# Autodesk Inventor assembly: ensamblaje socket
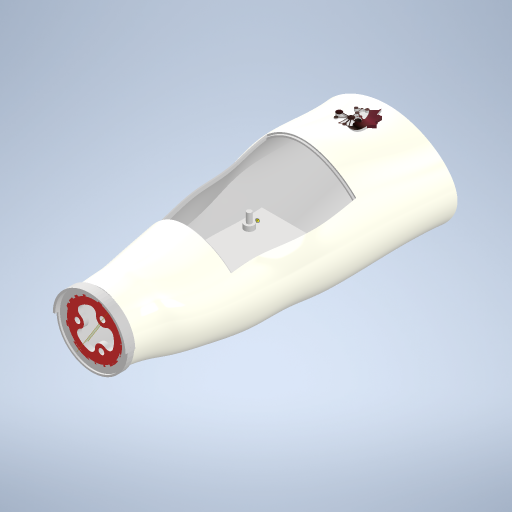
[picture p0: Inventor's stored thumbnail of the model, 512x512]
Saved by Autodesk Inventor 2024 (Build 280153000, 153)
## iProperties
Created: 2021-06-15
Part Number: ensamblaje socket
Document SubType Name: Assembly
Designer: ander
Author: ander
## Documents named in this file (4)
- X:\ensamblaje socket.iam
- X:\Forearm\protesis_antebrazo.ipt
- X:\Palm\palm_socket_connector.ipt
- X:\Forearm\socket_extension.ipt
## Components (3 placed, 3 different names)
1. protesis_antebrazo:1 — Insert:1, Angle:1, Angle:2
2. palm_socket_connector:1 — Insert:1, Angle:1, Insert:2
3. socket_extension:1 — Insert:2, Angle:2
## Relationships (4: Insert 2, Angle 2)
- Insert:1: protesis_antebrazo:1 ↔ palm_socket_connector:1
- Angle:1 (0 deg): protesis_antebrazo:1 ↔ palm_socket_connector:1
- Insert:2: palm_socket_connector:1 ↔ socket_extension:1
- Angle:2 (122.16 deg): protesis_antebrazo:1 ↔ socket_extension:1
